# Autodesk Inventor assembly: TVC assembly
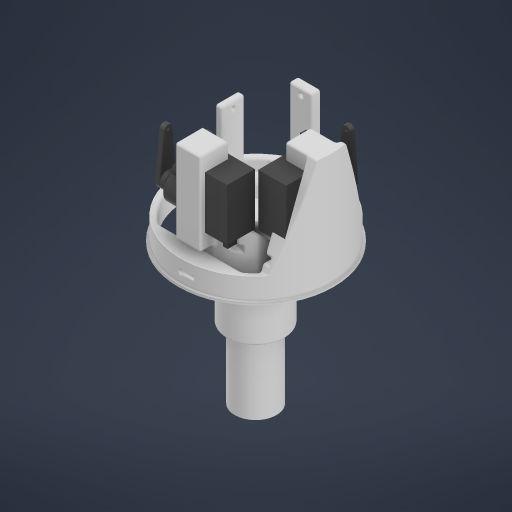
[picture p0: Inventor's stored thumbnail of the model, 512x512]
Saved by Autodesk Inventor 2024 (Build 280153000, 153)
## iProperties
Created: 2025-01-01
Part Number: TVC assembly
Document SubType Name: Assembly
Designer: huj31
Author: huj31
## Documents named in this file (7)
- C:\Users\huj31\OneDrive\Documents\__ school\Capstone\CAD\TVC assembly.iam
- C:\Users\huj31\OneDrive\Documents\__ school\Capstone\CAD\bt80tube.ipt
- C:\Users\huj31\OneDrive\Documents\__ school\Capstone\CAD\engine casing.ipt
- C:\Users\huj31\OneDrive\Documents\__ school\Capstone\CAD\middle gimbal.ipt
- C:\Users\huj31\OneDrive\Documents\__ school\Capstone\CAD\stationary ring.ipt
- C:\Users\huj31\OneDrive\Documents\__ school\Capstone\CAD\Servo.iam
- C:\Users\huj31\OneDrive\Documents\__ school\Capstone\CAD\18mm engine.ipt
## Components (7 placed, 6 different names)
1. bt80tube:1 — Flush:3, Mate:6
2. engine casing:1 — Mate:7, Mate:11, Mate:16, Flush:4
3. middle gimbal:1 — Mate:4, Mate:5, Mate:7, Mate:8, Mate:11, Mate:18, Mate:22
4. stationary ring:1 — Mate:4, Mate:5, Flush:3, Mate:6, Mate:19, Mate:20, Mate:21
5. Servo:5 [sub-assembly] — Mate:19, Mate:20, Mate:21
6. Servo:6 [sub-assembly] — Mate:8, Mate:18, Mate:22
7. 18mm engine:1 — Mate:16, Flush:4
## Relationships (14: Mate 12, Flush 2)
- Mate:4: middle gimbal:1 ↔ stationary ring:1
- Mate:5 (0.5 mm): middle gimbal:1 ↔ stationary ring:1
- Flush:3: bt80tube:1 ↔ stationary ring:1
- Mate:6: bt80tube:1 ↔ stationary ring:1
- Mate:7 (0.5 mm): engine casing:1 ↔ middle gimbal:1
- Mate:8: middle gimbal:1 ↔ Servo:6
- Mate:11: engine casing:1 ↔ middle gimbal:1
- Mate:16: engine casing:1 ↔ 18mm engine:1
- Flush:4 (5 mm): engine casing:1 ↔ 18mm engine:1
- Mate:18: middle gimbal:1 ↔ Servo:6
- Mate:19: stationary ring:1 ↔ Servo:5
- Mate:20: stationary ring:1 ↔ Servo:5
- Mate:21: stationary ring:1 ↔ Servo:5
- Mate:22: middle gimbal:1 ↔ Servo:6
